# Autodesk Inventor assembly: Bin_Assembly_IAM
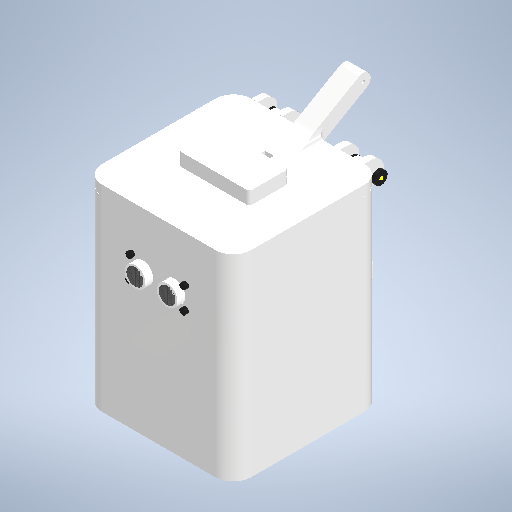
[picture p0: Inventor's stored thumbnail of the model, 512x512]
Saved by Autodesk Inventor 2025.2 (Build 292293000, 293)
## iProperties
Created: 2025-08-17
Part Number: Bin_Assembly_IAM
Document SubType Name: Assembly
Designer: Alan Rodrigues
Author: Alan Rodrigues
## Documents named in this file (9)
- C:\Users\Alan Rodrigues\Documents\SmartBin-Cad\Assembly\Bin_Assembly_IAM.iam
- C:\Users\Alan Rodrigues\Documents\Inventor\Orgulho_SESI.ipt
- C:\Users\Alan Rodrigues\Documents\[4145] TowerPro SG90 Mini Servo-SunRobotics_in-Sg90\[4145] TowerPro SG90 Mini Servo-SunRobotics_in-Sg90\[4145] TowerPro SG90 Mini Servo-SunRobotics_in-Sg90.iam
- C:\Users\Alan Rodrigues\Documents\HC-SR04\HC-SR04\HC-SR04.ipt
- C:\Users\Alan Rodrigues\Documents\Trava.ipt
- C:\Users\Alan Rodrigues\Documents\Travador.ipt
- C:\Users\Alan Rodrigues\Documents\Trava_Espaço.ipt
- C:\Users\Alan Rodrigues\Documents\Trava_Sensor.ipt
- C:\Users\Alan Rodrigues\Documents\Trava_Servo.ipt
## Components (22 placed, 8 different names)
1. Orgulho_SESI:1 — Ângulo:1, Ângulo:2, Inserir:1, Inserir:2, Inserir:3, Inserir:8, Inserir:9, Inserir:10, Inserir:11, Inserir:12, Inserir:13, Inserir:15, Inserir:16, Inserir:17, Inserir:18, Inserir:19, Inserir:20, Inserir:21, Inserir:22, Inserir:23, Inserir:24, Inserir:25
2. [4145] TowerPro SG90 Mini Servo-SunRobotics_in-Sg90:1 [sub-assembly] — Ângulo:1, Ângulo:2, Inserir:1
3. HC-SR04:1 — Inserir:2
4. HC-SR04:2 — Inserir:3
5. Trava_Espaço:2 — Inserir:9
6. Trava_Espaço:6 — Inserir:10
7. Trava_Espaço:7 — Inserir:11
8. Trava_Espaço:8 — Inserir:8
9. Trava:1 — Inserir:13
10. Trava:2 — Inserir:12, Inserir:14
11. Travador:1 — Inserir:14
12. Travador:2 — Inserir:15
13. Trava_Sensor:1 — Inserir:17
14. Trava_Sensor:2 — Inserir:18
15. Trava_Sensor:3 — Inserir:23
16. Trava_Sensor:4 — Inserir:21
17. Trava_Sensor:5 — Inserir:19
18. Trava_Sensor:6 — Inserir:20
19. Trava_Sensor:7 — Inserir:22
20. Trava_Sensor:8 — Inserir:16
21. Trava_Servo:1 — Inserir:25
22. Trava_Servo:2 — Inserir:24
## Relationships (23: Insert 21, Angle 2)
- Ângulo:1 [Angle] (180 deg): Orgulho_SESI:1 ↔ [4145] TowerPro SG90 Mini Servo-SunRobotics_in-Sg90:1
- Ângulo:2 [Angle] (180 deg): Orgulho_SESI:1 ↔ [4145] TowerPro SG90 Mini Servo-SunRobotics_in-Sg90:1
- Inserir:1: Orgulho_SESI:1 ↔ [4145] TowerPro SG90 Mini Servo-SunRobotics_in-Sg90:1
- Inserir:2 (-8 mm): Orgulho_SESI:1 ↔ HC-SR04:1
- Inserir:3 (-8 mm): Orgulho_SESI:1 ↔ HC-SR04:2
- Inserir:8 (0.1 mm): Orgulho_SESI:1 ↔ Trava_Espaço:8
- Inserir:9 (0.1 mm): Orgulho_SESI:1 ↔ Trava_Espaço:2
- Inserir:10 (0.1 mm): Orgulho_SESI:1 ↔ Trava_Espaço:6
- Inserir:11 (0.1 mm): Orgulho_SESI:1 ↔ Trava_Espaço:7
- Inserir:12 (-24.5 mm): Orgulho_SESI:1 ↔ Trava:2
- Inserir:13 (-24.5 mm): Orgulho_SESI:1 ↔ Trava:1
- Inserir:14 (-10 mm): Trava:2 ↔ Travador:1
- Inserir:15 (-10 mm): Orgulho_SESI:1 ↔ Travador:2
- Inserir:16 (-8 mm): Orgulho_SESI:1 ↔ Trava_Sensor:8
- Inserir:17 (-8 mm): Orgulho_SESI:1 ↔ Trava_Sensor:1
- Inserir:18 (-8 mm): Orgulho_SESI:1 ↔ Trava_Sensor:2
- Inserir:19 (-8 mm): Orgulho_SESI:1 ↔ Trava_Sensor:5
- Inserir:20 (-8 mm): Orgulho_SESI:1 ↔ Trava_Sensor:6
- Inserir:21 (-8 mm): Orgulho_SESI:1 ↔ Trava_Sensor:4
- Inserir:22 (-8 mm): Orgulho_SESI:1 ↔ Trava_Sensor:7
- Inserir:23 (-8 mm): Orgulho_SESI:1 ↔ Trava_Sensor:3
- Inserir:24 (-9 mm): Orgulho_SESI:1 ↔ Trava_Servo:2
- Inserir:25 (-9 mm): Orgulho_SESI:1 ↔ Trava_Servo:1
